(part 1 of 4)
# Autodesk Inventor assembly: ASSEMBLY_Main
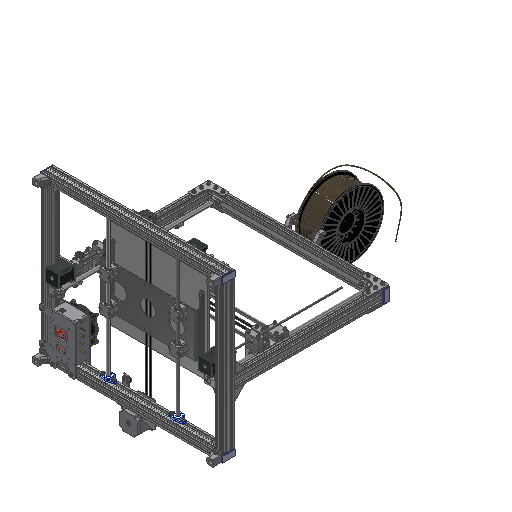
[picture p0: Inventor's stored thumbnail of the model, 512x512]
Saved by Autodesk Inventor 2026.1 (Build 301233000, 233)
## iProperties
Created: 2017-05-10
Part Number: ASSEMBLY_Main
Material: Ogólny
Document SubType Name: Assembly
Designer: Andrzej
Author: Andrzej
## Documents named in this file (88)
- C:\Users\Andrzej\OneDrive\_DRIVE_SYNCH_FILES\__ BYTECHLAB PROJECTS\MECH - FDM 3D Printer - TREX-300\MCAD\1_REV1\ASSEMBLY_MAIN_REVA\ASSEMBLY_Main.iam
- C:\Users\Andrzej\OneDrive\_DRIVE_SYNCH_FILES\__ BYTECHLAB PROJECTS\MECH - FDM 3D Printer - TREX-300\MCAD\1_REV1\ASSEMBLY_MAIN_REVA\LC_ALU_3mm_Top_Beam_Mounting_Bracket.ipt
- C:\Users\Andrzej\OneDrive\_DRIVE_SYNCH_FILES\__ BYTECHLAB PROJECTS\MECH - FDM 3D Printer - TREX-300\MCAD\1_REV1\__COTS_PARTS\COTS_GENERIC_20x40mm_alu_extrusion_460mm.ipt
- C:\Users\Andrzej\OneDrive\_DRIVE_SYNCH_FILES\__ BYTECHLAB PROJECTS\MECH - FDM 3D Printer - TREX-300\MCAD\1_REV1\__COTS_PARTS\COTS_GENERIC_20x40mm_alu_extrusion_560mm.ipt
- C:\Users\Andrzej\OneDrive\_DRIVE_SYNCH_FILES\__ BYTECHLAB PROJECTS\MECH - FDM 3D Printer - TREX-300\MCAD\1_REV1\__COTS_PARTS\COTS_GENERIC_20x40_Alu_Extrusion_Endcap.ipt
- C:\Users\Andrzej\OneDrive\_DRIVE_SYNCH_FILES\__ BYTECHLAB PROJECTS\MECH - FDM 3D Printer - TREX-300\MCAD\1_REV1\__COTS_PARTS\COTS_GENERIC_20x20mm_Angle_Bracket.ipt
- C:\Users\Andrzej\OneDrive\_DRIVE_SYNCH_FILES\__ BYTECHLAB PROJECTS\MECH - FDM 3D Printer - TREX-300\MCAD\1_REV1\ASSEMBLY_MAIN_REVA\CUT_STEEL_12mmx495mm_Linear_Shaft.ipt
- C:\Users\Andrzej\OneDrive\_DRIVE_SYNCH_FILES\__ BYTECHLAB PROJECTS\MECH - FDM 3D Printer - TREX-300\MCAD\1_REV1\ASSEMBLY_MAIN_REVA\CUT_STEEL_10mmx457mm_Linear_Shaft.ipt
- C:\Users\Andrzej\OneDrive\_DRIVE_SYNCH_FILES\__ BYTECHLAB PROJECTS\MECH - FDM 3D Printer - TREX-300\MCAD\1_REV1\ASSEMBLY_MAIN_REVA\LCBN_STEEL_3mm_Y_Axis_Heatbed_Baseplate.ipt
- C:\Users\Andrzej\OneDrive\_DRIVE_SYNCH_FILES\__ BYTECHLAB PROJECTS\MECH - FDM 3D Printer - TREX-300\MCAD\1_REV1\ASSEMBLY_MAIN_REVA\CNCM_ALU_6mm_Heatbed.ipt
- C:\Users\Andrzej\OneDrive\_DRIVE_SYNCH_FILES\__ BYTECHLAB PROJECTS\MECH - FDM 3D Printer - TREX-300\MCAD\1_REV1\ASSEMBLY_MAIN_REVA\CUT_STEEL_10mmx516mm_Linear_Shaft.ipt
- C:\Users\Andrzej\OneDrive\_DRIVE_SYNCH_FILES\__ BYTECHLAB PROJECTS\MECH - FDM 3D Printer - TREX-300\MCAD\1_REV1\ASSEMBLY_MAIN_REVA\LCBN_ALU_2mm_Y_Axis_Motor_Mount.ipt
- C:\Users\Andrzej\OneDrive\_DRIVE_SYNCH_FILES\__ BYTECHLAB PROJECTS\MECH - FDM 3D Printer - TREX-300\MCAD\1_REV1\ASSEMBLY_MAIN_REVA\3DP_ABS_Feet.ipt
- C:\Users\Andrzej\OneDrive\_DRIVE_SYNCH_FILES\__ BYTECHLAB PROJECTS\MECH - FDM 3D Printer - TREX-300\MCAD\1_REV1\ASSEMBLY_MAIN_REVA\3DP_ABS_Feet_MIR.ipt
- C:\Users\Andrzej\OneDrive\_DRIVE_SYNCH_FILES\__ BYTECHLAB PROJECTS\MECH - FDM 3D Printer - TREX-300\MCAD\1_REV1\ASSEMBLY_MAIN_REVA\3DP_ABS_Z_Axis_Endstop_Mount.ipt
- C:\Users\Andrzej\OneDrive\_DRIVE_SYNCH_FILES\__ BYTECHLAB PROJECTS\MECH - FDM 3D Printer - TREX-300\MCAD\1_REV1\__COTS_PARTS\COTS_GENERIC_Endstop.ipt
- C:\Users\Andrzej\OneDrive\_DRIVE_SYNCH_FILES\__ BYTECHLAB PROJECTS\MECH - FDM 3D Printer - TREX-300\MCAD\1_REV1\ASSEMBLY_MAIN_REVA\CNCM_ALU_3mm_Y_Axis_Idler_Stiffener_Side.ipt
- C:\Users\Andrzej\OneDrive\_DRIVE_SYNCH_FILES\__ BYTECHLAB PROJECTS\MECH - FDM 3D Printer - TREX-300\MCAD\1_REV1\ASSEMBLY_MAIN_REVA\LCBN_ALU_3mm_Y_Axis_Idler_Stiffener_Top.ipt
- C:\Users\Andrzej\OneDrive\_DRIVE_SYNCH_FILES\__ BYTECHLAB PROJECTS\MECH - FDM 3D Printer - TREX-300\MCAD\1_REV1\ASSEMBLY_MAIN_REVA\3DP_ABS_Y_Axis_Endstop_Mount.ipt
- C:\Users\Andrzej\OneDrive\_DRIVE_SYNCH_FILES\__ BYTECHLAB PROJECTS\MECH - FDM 3D Printer - TREX-300\MCAD\1_REV1\__COTS_PARTS\COTS_GENERIC_Bearing_12x5x5.ipt
- C:\Users\Andrzej\OneDrive\_DRIVE_SYNCH_FILES\__ BYTECHLAB PROJECTS\MECH - FDM 3D Printer - TREX-300\MCAD\1_REV1\__COTS_PARTS\COTS_GENERIC_Y_Axis_Timing_Belt.ipt
- C:\Users\Andrzej\OneDrive\_DRIVE_SYNCH_FILES\__ BYTECHLAB PROJECTS\MECH - FDM 3D Printer - TREX-300\MCAD\1_REV1\ASSEMBLY_MAIN_REVA\3DP_ABS_Y_Axis_Linear_Bearing_Mount_Top.ipt
- C:\Users\Andrzej\OneDrive\_DRIVE_SYNCH_FILES\__ BYTECHLAB PROJECTS\MECH - FDM 3D Printer - TREX-300\MCAD\1_REV1\ASSEMBLY_MAIN_REVA\3DP_ABS_Y_Axis_Linear_Bearing_Mount_Bottom.ipt
- C:\Users\Andrzej\OneDrive\_DRIVE_SYNCH_FILES\__ BYTECHLAB PROJECTS\MECH - FDM 3D Printer - TREX-300\MCAD\1_REV1\ASSEMBLY_MAIN_REVA\3DP_ABS_Y_Axis_Belt_Mount_Spacer.ipt
- C:\Users\Andrzej\OneDrive\_DRIVE_SYNCH_FILES\__ BYTECHLAB PROJECTS\MECH - FDM 3D Printer - TREX-300\MCAD\1_REV1\ASSEMBLY_MAIN_REVA\LC_ALU_4mm_X_End_Motor_Side.ipt
- C:\Users\Andrzej\OneDrive\_DRIVE_SYNCH_FILES\__ BYTECHLAB PROJECTS\MECH - FDM 3D Printer - TREX-300\MCAD\1_REV1\ASSEMBLY_MAIN_REVA\3DP_ABS_X_Axis_Linear_Shaft_Clamp_Base.ipt
- C:\Users\Andrzej\OneDrive\_DRIVE_SYNCH_FILES\__ BYTECHLAB PROJECTS\MECH - FDM 3D Printer - TREX-300\MCAD\1_REV1\ASSEMBLY_MAIN_REVA\LC_ALU_4mm_X_End_Bearing_Side.ipt
- C:\Users\Andrzej\OneDrive\_DRIVE_SYNCH_FILES\__ BYTECHLAB PROJECTS\MECH - FDM 3D Printer - TREX-300\MCAD\1_REV1\ASSEMBLY_MAIN_REVA\3DP_ABS_X_Axis_Linear_Shaft_Clamp_Top.ipt
- C:\Users\Andrzej\OneDrive\_DRIVE_SYNCH_FILES\__ BYTECHLAB PROJECTS\MECH - FDM 3D Printer - TREX-300\MCAD\1_REV1\ASSEMBLY_MAIN_REVA\3DP_ABS_X_Axis_Linear_Shaft_Clamp_Bottom.ipt
- C:\Users\Andrzej\OneDrive\_DRIVE_SYNCH_FILES\__ BYTECHLAB PROJECTS\MECH - FDM 3D Printer - TREX-300\MCAD\1_REV1\ASSEMBLY_MAIN_REVA\3DP_PLA_Controller_Case_Bottom.ipt
- C:\Users\Andrzej\OneDrive\_DRIVE_SYNCH_FILES\__ BYTECHLAB PROJECTS\MECH - FDM 3D Printer - TREX-300\MCAD\1_REV1\ASSEMBLY_MAIN_REVA\3DP_PLA_Controller_Case_Side_Wall_Longer.ipt
- C:\Users\Andrzej\OneDrive\_DRIVE_SYNCH_FILES\__ BYTECHLAB PROJECTS\MECH - FDM 3D Printer - TREX-300\MCAD\1_REV1\ASSEMBLY_MAIN_REVA\3DP_PLA_Controller_Case_Side_Wall_Shorter.ipt
- C:\Users\Andrzej\OneDrive\_DRIVE_SYNCH_FILES\__ BYTECHLAB PROJECTS\MECH - FDM 3D Printer - TREX-300\MCAD\1_REV1\ASSEMBLY_MAIN_REVA\3DP_PLA_Controller_Case_Top.ipt
- C:\Users\Andrzej\OneDrive\_DRIVE_SYNCH_FILES\__ BYTECHLAB PROJECTS\MECH - FDM 3D Printer - TREX-300\MCAD\1_REV1\ASSEMBLY_MAIN_REVA\3DP_PLA_Controller_Case_Fan_Grill.ipt
- C:\Users\Andrzej\OneDrive\_DRIVE_SYNCH_FILES\__ BYTECHLAB PROJECTS\MECH - FDM 3D Printer - TREX-300\MCAD\1_REV1\ASSEMBLY_MAIN_REVA\3DP_PLA_Filament_Spool_Rollers.ipt
- C:\Users\Andrzej\OneDrive\_DRIVE_SYNCH_FILES\__ BYTECHLAB PROJECTS\MECH - FDM 3D Printer - TREX-300\MCAD\1_REV1\__COTS_PARTS\COTS_GENERIC_Bearing_19x5x6.ipt
- C:\Users\Andrzej\OneDrive\_DRIVE_SYNCH_FILES\__ BYTECHLAB PROJECTS\MECH - FDM 3D Printer - TREX-300\MCAD\1_REV1\__COTS_PARTS\COTS_GENERIC_1_75mm_Filament_Spool.ipt
- C:\Users\Andrzej\OneDrive\_DRIVE_SYNCH_FILES\__ BYTECHLAB PROJECTS\MECH - FDM 3D Printer - TREX-300\MCAD\1_REV1\ASSEMBLY_MAIN_REVA\3DP_ABS_X_Axis_Endstop_Mount.ipt
- C:\Users\Andrzej\OneDrive\_DRIVE_SYNCH_FILES\__ BYTECHLAB PROJECTS\MECH - FDM 3D Printer - TREX-300\MCAD\1_REV1\ASSEMBLY_MAIN_REVA\3DP_ABS_X_Axis_Linear_Shaft_Clamp_Bottom_With_Endstop_Screw.ipt
- C:\Users\Andrzej\OneDrive\_DRIVE_SYNCH_FILES\__ BYTECHLAB PROJECTS\MECH - FDM 3D Printer - TREX-300\MCAD\1_REV1\ASSEMBLY_MAIN_REVA\3DP_ABS_Z_Axis_Screw_Nut_Mount.ipt
- C:\Users\Andrzej\OneDrive\_DRIVE_SYNCH_FILES\__ BYTECHLAB PROJECTS\MECH - FDM 3D Printer - TREX-300\MCAD\1_REV1\__COTS_PARTS\COTS_GENERIC_M6x350mm_Z_Axis_Screw.ipt
- C:\Users\Andrzej\OneDrive\_DRIVE_SYNCH_FILES\__ BYTECHLAB PROJECTS\MECH - FDM 3D Printer - TREX-300\MCAD\1_REV1\__COTS_PARTS\COTS_GENERIC_Z_Axis_M6_Screw_Nut.ipt
- C:\Users\Andrzej\OneDrive\_DRIVE_SYNCH_FILES\__ BYTECHLAB PROJECTS\MECH - FDM 3D Printer - TREX-300\MCAD\1_REV1\ASSEMBLY_MAIN_REVA\LC_ALU_4mm_Z_Axis_Motor_Mount.ipt
- C:\Users\Andrzej\OneDrive\_DRIVE_SYNCH_FILES\__ BYTECHLAB PROJECTS\MECH - FDM 3D Printer - TREX-300\MCAD\1_REV1\ASSEMBLY_MAIN_REVA\3DP_ABS_Z_Axis_Screw_Coupler.ipt
- C:\Users\Andrzej\OneDrive\_DRIVE_SYNCH_FILES\__ BYTECHLAB PROJECTS\MECH - FDM 3D Printer - TREX-300\MCAD\1_REV1\__COTS_PARTS\COTS_GENERIC_MXL_Pulley_X_Axis.ipt
- C:\Users\Andrzej\OneDrive\_DRIVE_SYNCH_FILES\__ BYTECHLAB PROJECTS\MECH - FDM 3D Printer - TREX-300\MCAD\1_REV1\__COTS_PARTS\COTS_GENERIC_Bearing_13x4x5.ipt
- C:\Users\Andrzej\OneDrive\_DRIVE_SYNCH_FILES\__ BYTECHLAB PROJECTS\MECH - FDM 3D Printer - TREX-300\MCAD\1_REV1\ASSEMBLY_MAIN_REVA\3DP_ABS_Cable_Pipe_Mount.ipt
- C:\Users\Andrzej\OneDrive\_DRIVE_SYNCH_FILES\__ BYTECHLAB PROJECTS\MECH - FDM 3D Printer - TREX-300\MCAD\1_REV1\ASSEMBLY_MAIN_REVA\3DP_ABS_X_End_Bearing_Mount.ipt
- C:\Users\Andrzej\OneDrive\_DRIVE_SYNCH_FILES\__ BYTECHLAB PROJECTS\MECH - FDM 3D Printer - TREX-300\MCAD\1_REV1\__COTS_PARTS\COTS_GENERIC_X_Axis_Timing_Belt.ipt
- C:\Users\Andrzej\OneDrive\_DRIVE_SYNCH_FILES\__ BYTECHLAB PROJECTS\MECH - FDM 3D Printer - TREX-300\MCAD\1_REV1\ASSEMBLY_MAIN_REVA\3DP_ABS_X_Axis_Motor_Spacer.ipt
- C:\Users\Andrzej\OneDrive\_DRIVE_SYNCH_FILES\__ BYTECHLAB PROJECTS\MECH - FDM 3D Printer - TREX-300\MCAD\1_REV1\ASSEMBLY_X_AXIS_CARRIAGE_AND_EXTRUDER\ASSEMBLY_X_Axis_Carriage_and_Extruder_Belt_Gearbox.iam
- C:\Users\Andrzej\OneDrive\_DRIVE_SYNCH_FILES\__ BYTECHLAB PROJECTS\MECH - FDM 3D Printer - TREX-300\MCAD\1_REV1\__COTS_PARTS\COTS_GENERIC_RAMPS_14_Ardunio_Mega\COTS_GENERIC_RAMPS_14_Ardunio_Mega.iam
- C:\Users\Andrzej\OneDrive\_DRIVE_SYNCH_FILES\__ BYTECHLAB PROJECTS\MECH - FDM 3D Printer - TREX-300\MCAD\1_REV1\__COTS_PARTS\COTS_GENERIC_80mm_fan\COTS_GENERIC_80mm_fan.iam
- C:\Users\Andrzej\OneDrive\_DRIVE_SYNCH_FILES\__ BYTECHLAB PROJECTS\MECH - FDM 3D Printer - TREX-300\MCAD\1_REV1\__CONTENT_CENTER_PARTS\en-US\DIN 125-1  A\DIN 125 - A 5,3.ipt
- C:\Users\Andrzej\OneDrive\_DRIVE_SYNCH_FILES\__ BYTECHLAB PROJECTS\MECH - FDM 3D Printer - TREX-300\MCAD\1_REV1\__CONTENT_CENTER_PARTS\en-US\DIN 912\DIN 912 - M5 x 0,8 x 30 x 22.ipt
- C:\Users\Andrzej\OneDrive\_DRIVE_SYNCH_FILES\__ BYTECHLAB PROJECTS\MECH - FDM 3D Printer - TREX-300\MCAD\1_REV1\__CONTENT_CENTER_PARTS\en-US\DIN 912\DIN 912 - M5 x 0,8 x 50 x 22.ipt
- C:\Users\Andrzej\OneDrive\_DRIVE_SYNCH_FILES\__ BYTECHLAB PROJECTS\MECH - FDM 3D Printer - TREX-300\MCAD\1_REV1\__CONTENT_CENTER_PARTS\en-US\DIN 125-1  A\DIN 125 - A 3,2.ipt
- C:\Users\Andrzej\OneDrive\_DRIVE_SYNCH_FILES\__ BYTECHLAB PROJECTS\MECH - FDM 3D Printer - TREX-300\MCAD\1_REV1\__CONTENT_CENTER_PARTS\en-US\ISO 7380-1\ISO 7380-1 - M3 x 12.ipt
- C:\Users\Andrzej\OneDrive\_DRIVE_SYNCH_FILES\__ BYTECHLAB PROJECTS\MECH - FDM 3D Printer - TREX-300\MCAD\1_REV1\__CONTENT_CENTER_PARTS\en-US\ISO 7380-1\ISO 7380-1 - M3 x 30.ipt
- C:\Users\Andrzej\OneDrive\_DRIVE_SYNCH_FILES\__ BYTECHLAB PROJECTS\MECH - FDM 3D Printer - TREX-300\MCAD\1_REV1\__CONTENT_CENTER_PARTS\en-US\DIN 934\DIN 934 - M3 x 0,5.ipt
- C:\Users\Andrzej\OneDrive\_DRIVE_SYNCH_FILES\__ BYTECHLAB PROJECTS\MECH - FDM 3D Printer - TREX-300\MCAD\1_REV1\__CONTENT_CENTER_PARTS\en-US\ISO 7380-1\ISO 7380-1 - M3 x 20.ipt
- C:\Users\Andrzej\OneDrive\_DRIVE_SYNCH_FILES\__ BYTECHLAB PROJECTS\MECH - FDM 3D Printer - TREX-300\MCAD\1_REV1\__CONTENT_CENTER_PARTS\en-US\DIN 912\DIN 912 - M3 x 0,5 x 20 x 18,75.ipt
- C:\Users\Andrzej\OneDrive\_DRIVE_SYNCH_FILES\__ BYTECHLAB PROJECTS\MECH - FDM 3D Printer - TREX-300\MCAD\1_REV1\__CONTENT_CENTER_PARTS\en-US\DIN 125-1  A\DIN 125 - A 4,3.ipt
- C:\Users\Andrzej\OneDrive\_DRIVE_SYNCH_FILES\__ BYTECHLAB PROJECTS\MECH - FDM 3D Printer - TREX-300\MCAD\1_REV1\__CONTENT_CENTER_PARTS\en-US\DIN 912\DIN 912 - M4 x 0,7 x 30 x 20.ipt
- C:\Users\Andrzej\OneDrive\_DRIVE_SYNCH_FILES\__ BYTECHLAB PROJECTS\MECH - FDM 3D Printer - TREX-300\MCAD\1_REV1\__CONTENT_CENTER_PARTS\en-US\DIN 934\DIN 934 - M4 x 0,7.ipt
- C:\Users\Andrzej\OneDrive\_DRIVE_SYNCH_FILES\__ BYTECHLAB PROJECTS\MECH - FDM 3D Printer - TREX-300\MCAD\1_REV1\__COTS_PARTS\COTS_GENERIC_20x20_M3_Nut.ipt
- C:\Users\Andrzej\OneDrive\_DRIVE_SYNCH_FILES\__ BYTECHLAB PROJECTS\MECH - FDM 3D Printer - TREX-300\MCAD\1_REV1\__CONTENT_CENTER_PARTS\en-US\DIN 912\DIN 912 - M3 x 0,5 x 16 x 14,75.ipt
- C:\Users\Andrzej\OneDrive\_DRIVE_SYNCH_FILES\__ BYTECHLAB PROJECTS\MECH - FDM 3D Printer - TREX-300\MCAD\1_REV1\__CONTENT_CENTER_PARTS\en-US\DIN 912\DIN 912 - M5 x 0,8 x 25 x 23.ipt
- C:\Users\Andrzej\OneDrive\_DRIVE_SYNCH_FILES\__ BYTECHLAB PROJECTS\MECH - FDM 3D Printer - TREX-300\MCAD\1_REV1\__CONTENT_CENTER_PARTS\en-US\DIN 934\DIN 934 - M5 x 0,8.ipt
- C:\Users\Andrzej\OneDrive\_DRIVE_SYNCH_FILES\__ BYTECHLAB PROJECTS\MECH - FDM 3D Printer - TREX-300\MCAD\1_REV1\__CONTENT_CENTER_PARTS\en-US\DIN 912\DIN 912 - M5 x 0,8 x 8 x 6.ipt
- C:\Users\Andrzej\OneDrive\_DRIVE_SYNCH_FILES\__ BYTECHLAB PROJECTS\MECH - FDM 3D Printer - TREX-300\MCAD\1_REV1\__CONTENT_CENTER_PARTS\en-US\DIN 912\DIN 912 - M5 x 0,8 x 12 x 10.ipt
- C:\Users\Andrzej\OneDrive\_DRIVE_SYNCH_FILES\__ BYTECHLAB PROJECTS\MECH - FDM 3D Printer - TREX-300\MCAD\1_REV1\__CONTENT_CENTER_PARTS\en-US\DIN 912\DIN 912 - M3 x 0,5 x 8 x 6,75.ipt
- C:\Users\Andrzej\OneDrive\_DRIVE_SYNCH_FILES\__ BYTECHLAB PROJECTS\MECH - FDM 3D Printer - TREX-300\MCAD\1_REV1\__CONTENT_CENTER_PARTS\en-US\DIN 7991(2)\DIN 7991 - M3x8.ipt
- C:\Users\Andrzej\OneDrive\_DRIVE_SYNCH_FILES\__ BYTECHLAB PROJECTS\MECH - FDM 3D Printer - TREX-300\MCAD\1_REV1\__CONTENT_CENTER_PARTS\en-US\DIN 912\DIN 912 - M4 x 0,7 x 40 x 20.ipt
- C:\Users\Andrzej\OneDrive\_DRIVE_SYNCH_FILES\__ BYTECHLAB PROJECTS\MECH - FDM 3D Printer - TREX-300\MCAD\1_REV1\__COTS_PARTS\COTS_GENERIC_NEMA17_25mm_shaft.ipt
- C:\Users\Andrzej\OneDrive\_DRIVE_SYNCH_FILES\__ BYTECHLAB PROJECTS\MECH - FDM 3D Printer - TREX-300\MCAD\1_REV1\__COTS_PARTS\COTS_GENERIC_SHF12_Linear_Rail_Mount\COTS_GENERIC_SHF12_Linear_Rail_Mount.iam
- C:\Users\Andrzej\OneDrive\_DRIVE_SYNCH_FILES\__ BYTECHLAB PROJECTS\MECH - FDM 3D Printer - TREX-300\MCAD\1_REV1\__COTS_PARTS\COTS_GENERIC_SK12_Linear_Rail_Mount\COTS_GENERIC_SK12_Linear_Rail_Mount.iam
- C:\Users\Andrzej\OneDrive\_DRIVE_SYNCH_FILES\__ BYTECHLAB PROJECTS\MECH - FDM 3D Printer - TREX-300\MCAD\1_REV1\__COTS_PARTS\COTS_GENERIC_NEMA23_Stepper_Motor\COTS_GENERIC_NEMA23_Stepper_Motor.iam
- C:\Users\Andrzej\OneDrive\_DRIVE_SYNCH_FILES\__ BYTECHLAB PROJECTS\MECH - FDM 3D Printer - TREX-300\MCAD\1_REV1\__COTS_PARTS\COTS_GENERIC_LM10UU_10mm_Linear_Bearing.ipt
- C:\Users\Andrzej\OneDrive\_DRIVE_SYNCH_FILES\__ BYTECHLAB PROJECTS\MECH - FDM 3D Printer - TREX-300\MCAD\1_REV1\__COTS_PARTS\COTS_GENERIC_SMA12GUU_Linear_Bearing_Block.ipt
- C:\Users\Andrzej\OneDrive\_DRIVE_SYNCH_FILES\__ BYTECHLAB PROJECTS\MECH - FDM 3D Printer - TREX-300\MCAD\1_REV1\__COTS_PARTS\COTS_GENERIC_SHF10_Linear_Rail_Mount.ipt
- C:\Users\Andrzej\OneDrive\_DRIVE_SYNCH_FILES\__ BYTECHLAB PROJECTS\MECH - FDM 3D Printer - TREX-300\MCAD\1_REV1\__COTS_PARTS\COTS_GENERIC_22x5_Washer.ipt
- C:\Users\Andrzej\OneDrive\_DRIVE_SYNCH_FILES\__ BYTECHLAB PROJECTS\MECH - FDM 3D Printer - TREX-300\MCAD\1_REV1\__CONTENT_CENTER_PARTS\en-US\DIN 912\DIN 912 - M4 x 0,7 x 8 x 6,25.ipt
- C:\Users\Andrzej\OneDrive\_DRIVE_SYNCH_FILES\__ BYTECHLAB PROJECTS\MECH - FDM 3D Printer - TREX-300\MCAD\1_REV1\__CONTENT_CENTER_PARTS\en-US\DIN 912\DIN 912 - M4 x 0,7 x 10 x 8,25.ipt
- C:\Users\Andrzej\OneDrive\_DRIVE_SYNCH_FILES\__ BYTECHLAB PROJECTS\MECH - FDM 3D Printer - TREX-300\MCAD\1_REV1\__CONTENT_CENTER_PARTS\en-US\DIN 912\DIN 912 - M5 x 0,8 x 10 x 8.ipt
- C:\Users\Andrzej\OneDrive\_DRIVE_SYNCH_FILES\__ BYTECHLAB PROJECTS\MECH - FDM 3D Printer - TREX-300\MCAD\1_REV1\__CONTENT_CENTER_PARTS\en-US\DIN 912\DIN 912 - M3 x 0,5 x 10 x 8,75.ipt
- C:\Users\Andrzej\OneDrive\_DRIVE_SYNCH_FILES\__ BYTECHLAB PROJECTS\MECH - FDM 3D Printer - TREX-300\MCAD\1_REV1\__CONTENT_CENTER_PARTS\en-US\DIN 912\DIN 912 - M3 x 0,5 x 30 x 18.ipt
- C:\Users\Andrzej\OneDrive\_DRIVE_SYNCH_FILES\__ BYTECHLAB PROJECTS\MECH - FDM 3D Printer - TREX-300\MCAD\1_REV1\__CONTENT_CENTER_PARTS\en-US\ISO 10642(1)\ISO 10642 - M4 x  20.ipt
## Components (507 placed, 87 different names)
1. COTS_GENERIC_20x40mm_alu_extrusion_460mm:1 — Zestawiający:7, Równoległy:13, Równoległy:14, Zestawiający:9, Równoległy:17, Równoległy:18, Zestawiający:10, Równoległy:19, Równoległy:25, Równoległy:48, Zestawiający:28, Zestawiający:32, Zestawiający:34, Równoległy:52, Równoległy:53, Zestawiający:40, Równoległy:55, Równoległy:69, Równoległy:76, Zestawiający:152, Równoległy:129, Równoległy:134, Zestawiający:211, Równoległy:150, Zestawiający:232
2. COTS_GENERIC_20x40mm_alu_extrusion_460mm:2 — Zestawiający:8, Równoległy:15, Równoległy:16, Zestawiający:11, Równoległy:20, Równoległy:47, Zestawiający:27, Zestawiający:31, Zestawiający:33, Równoległy:51, Równoległy:54, Zestawiający:39, Równoległy:56, Zestawiający:64, Równoległy:71, Równoległy:73, Zestawiający:207, Równoległy:149
3. COTS_GENERIC_20x40mm_alu_extrusion_460mm:3 — Zestawiający:10, Równoległy:19, Zestawiający:12, Równoległy:21, Równoległy:22, Równoległy:25, Zestawiający:13, Równoległy:26, Równoległy:28, Zestawiający:24, Zestawiający:30, Równoległy:49, Równoległy:57, Zestawiający:84, Równoległy:81, Równoległy:136, Zestawiający:230, Zestawiający:231, Zestawiający:233, Zestawiający:234
4. COTS_GENERIC_20x40mm_alu_extrusion_460mm:4 — Zestawiający:11, Równoległy:20, Równoległy:23, Równoległy:24, Zestawiający:16, Równoległy:31, Równoległy:42, Zestawiający:26, Zestawiający:29, Równoległy:50, Równoległy:58
5. COTS_GENERIC_20x40mm_alu_extrusion_560mm:1 — Zestawiający:7, Równoległy:13, Równoległy:14, Zestawiający:8, Równoległy:15, Równoległy:16, Zestawiający:19, Zestawiający:21, Równoległy:34, Równoległy:35, Równoległy:43, Równoległy:44, Zestawiający:35, Zestawiający:36, Zestawiający:53, Zestawiający:54, Równoległy:59, Równoległy:60, Zestawiający:61, Zestawiający:62, Zestawiający:76, Równoległy:72, Zestawiający:82, Równoległy:75, Zestawiający:94, Równoległy:89, Równoległy:92, Równoległy:93, Równoległy:128, Równoległy:135
6. COTS_GENERIC_20x40mm_alu_extrusion_560mm:2 — Zestawiający:12, Równoległy:21, Równoległy:22, Równoległy:23, Równoległy:24, Zestawiający:14, Zestawiający:15, Równoległy:27, Równoległy:29, Równoległy:30, Równoległy:33, Zestawiający:17, Zestawiający:20, Równoległy:38, Równoległy:39, Równoległy:40, Równoległy:41, Zestawiający:41, Zestawiający:42, Zestawiający:47, Zestawiający:48, Zestawiający:164, Zestawiający:165, Zestawiający:176, Zestawiający:177, Równoległy:155, Mate:306, Mate:307, Flush:161, Flush:162, Mate:363, Mate:364
7. COTS_GENERIC_20x40mm_alu_extrusion_560mm:3 — Zestawiający:9, Równoległy:17, Równoległy:18, Zestawiający:18, Zestawiający:22, Równoległy:36, Równoległy:37, Równoległy:45, Równoległy:46, Zestawiający:37, Zestawiający:38, Zestawiający:55, Zestawiający:56, Równoległy:61, Równoległy:62, Zestawiający:79, Równoległy:70, Zestawiający:80, Zestawiający:81, Równoległy:74, Zestawiający:86, Zestawiający:87, Równoległy:84, Równoległy:85
8. LC_ALU_3mm_Top_Beam_Mounting_Bracket:1 — Zestawiający:13, Równoległy:28, Równoległy:29
9. LC_ALU_3mm_Top_Beam_Mounting_Bracket:2 — Zestawiający:14, Równoległy:26, Równoległy:27
10. LC_ALU_3mm_Top_Beam_Mounting_Bracket:3 — Zestawiający:15, Równoległy:30, Równoległy:31, Mate:328, Mate:329, Mate:330, Mate:331, Mate:332, Mate:333, Mate:334, Mate:335, Mate:336, Mate:337
11. LC_ALU_3mm_Top_Beam_Mounting_Bracket:4 — Zestawiający:16, Równoległy:33, Równoległy:42
12. COTS_GENERIC_20x40_Alu_Extrusion_Endcap:1 — Zestawiający:18, Równoległy:45, Równoległy:46
13. COTS_GENERIC_20x40_Alu_Extrusion_Endcap:2 — Zestawiający:17, Równoległy:40, Równoległy:41
14. COTS_GENERIC_20x40_Alu_Extrusion_Endcap:3 — Zestawiający:19, Równoległy:43, Równoległy:44
15. COTS_GENERIC_20x40_Alu_Extrusion_Endcap:4 — Zestawiający:20, Równoległy:38, Równoległy:39
16. COTS_GENERIC_20x40_Alu_Extrusion_Endcap:5 — Zestawiający:21, Równoległy:34, Równoległy:35
17. COTS_GENERIC_20x40_Alu_Extrusion_Endcap:6 — Zestawiający:22, Równoległy:36, Równoległy:37
18. COTS_GENERIC_20x20mm_Angle_Bracket:1 — Zestawiający:33, Zestawiający:37, Równoległy:54, Mate:499, Mate:521, Mate:522, Mate:524
19. COTS_GENERIC_20x20mm_Angle_Bracket:2 — Zestawiający:24, Równoległy:48, Zestawiający:218, Mate:475, Mate:483
20. COTS_GENERIC_20x20mm_Angle_Bracket:3 — Zestawiający:28, Zestawiający:30, Równoległy:49, Mate:479, Mate:487
21. COTS_GENERIC_20x20mm_Angle_Bracket:4 — Zestawiający:34, Zestawiający:38, Równoległy:53, Mate:501, Mate:502, Mate:504, Mate:523
22. COTS_GENERIC_20x20mm_Angle_Bracket:5 — Zestawiający:26, Równoległy:47, Zestawiający:217, Mate:473, Mate:474, Mate:476, Mate:481, Mate:482, Mate:484
23. COTS_GENERIC_20x20mm_Angle_Bracket:6 — Zestawiający:31, Zestawiający:36, Równoległy:51, Mate:497, Mate:498, Mate:500, Mate:525, Mate:526, Mate:528
24. COTS_GENERIC_20x20mm_Angle_Bracket:7 — Zestawiający:32, Zestawiający:35, Równoległy:52, Mate:503, Mate:527
25. COTS_GENERIC_20x20mm_Angle_Bracket:8 — Zestawiający:27, Zestawiający:29, Równoległy:50, Mate:477, Mate:478, Mate:480, Mate:485, Mate:486, Mate:488
26. COTS_GENERIC_SK12_Linear_Rail_Mount:1 [sub-assembly] — Zestawiający:40, Równoległy:55, Równoległy:57, Zestawiający:45, Mate:493, Mate:494, Mate:495, Mate:496
27. COTS_GENERIC_SK12_Linear_Rail_Mount:2 [sub-assembly] — Zestawiający:39, Równoległy:56, Równoległy:58, Zestawiający:43, Mate:489, Mate:490, Mate:491, Mate:492
28. COTS_GENERIC_SHF12_Linear_Rail_Mount:1 [sub-assembly] — Zestawiający:41, Zestawiający:44, Mate:363, Mate:369, Mate:371
29. COTS_GENERIC_SHF12_Linear_Rail_Mount:2 [sub-assembly] — Zestawiający:42, Zestawiający:46, Mate:364, Mate:365, Mate:366, Mate:367, Mate:368, Mate:370, Mate:372
30. CUT_STEEL_12mmx495mm_Linear_Shaft:1 — Zestawiający:45, Zestawiający:46, Zestawiający:47, Zestawiający:49, Zestawiający:50
31. CUT_STEEL_12mmx495mm_Linear_Shaft:2 — Zestawiający:43, Zestawiający:44, Zestawiający:48, Zestawiający:51, Zestawiający:52
32. COTS_GENERIC_SMA12GUU_Linear_Bearing_Block:1 — Zestawiający:52, Równoległy:66, Równoległy:67, Równoległy:79, Równoległy:113, Równoległy:114
33. COTS_GENERIC_SMA12GUU_Linear_Bearing_Block:2 — Zestawiający:50, Równoległy:65, Równoległy:67, Równoległy:79, Zestawiający:134, Równoległy:104, Równoległy:106, Równoległy:158
34. COTS_GENERIC_SMA12GUU_Linear_Bearing_Block:3 — Zestawiający:51, Równoległy:66, Równoległy:80, Zestawiający:143
35. COTS_GENERIC_SMA12GUU_Linear_Bearing_Block:4 — Zestawiający:49, Równoległy:65, Równoległy:80, Równoległy:105
36. COTS_GENERIC_RAMPS_14_Ardunio_Mega:1 [sub-assembly] — Zestawiający:156, Zestawiający:191
37. ASSEMBLY_X_Axis_Carriage_and_Extruder_Belt_Gearbox:1 [sub-assembly] — Zestawiający:141, Zestawiający:142
38. COTS_GENERIC_SHF10_Linear_Rail_Mount:1 — Zestawiający:54, Zestawiający:58, Równoległy:60, Mate:541, Mate:543
39. COTS_GENERIC_SHF10_Linear_Rail_Mount:2 — Zestawiający:53, Zestawiający:57, Równoległy:59, Mate:537, Mate:538, Mate:539, Mate:540, Mate:542, Mate:544
40. COTS_GENERIC_SHF10_Linear_Rail_Mount:3 — Zestawiający:55, Zestawiający:59, Równoległy:61, Mate:533, Mate:535
41. COTS_GENERIC_SHF10_Linear_Rail_Mount:4 — Zestawiający:56, Zestawiający:60, Równoległy:62, Mate:529, Mate:530, Mate:531, Mate:532, Mate:534, Mate:536
42. CUT_STEEL_10mmx457mm_Linear_Shaft:1 — Zestawiający:57, Zestawiający:60, Zestawiający:61, Zestawiający:63, Zestawiający:67, Zestawiający:68, Zestawiający:71
43. CUT_STEEL_10mmx457mm_Linear_Shaft:2 — Zestawiający:58, Zestawiający:59, Zestawiający:62, Zestawiający:63, Zestawiający:64, Zestawiający:65, Zestawiający:66, Zestawiający:72, Zestawiający:125
44. COTS_GENERIC_LM10UU_10mm_Linear_Bearing:1 — Zestawiający:66, Zestawiający:128
45. COTS_GENERIC_LM10UU_10mm_Linear_Bearing:2 — Zestawiający:65, Zestawiający:126
46. COTS_GENERIC_LM10UU_10mm_Linear_Bearing:3 — Zestawiający:67, Zestawiający:124, Zestawiający:127
47. COTS_GENERIC_LM10UU_10mm_Linear_Bearing:4 — Zestawiający:68, Zestawiający:129
48. LCBN_STEEL_3mm_Y_Axis_Heatbed_Baseplate:1 — Zestawiający:71, Zestawiający:72, Zestawiający:73, Równoległy:63, Równoległy:64, Zestawiający:108, Zestawiający:109, Zestawiający:110, Zestawiający:111, Zestawiający:112, Zestawiający:113, Zestawiający:114, Zestawiający:115, Zestawiający:116, Zestawiający:117, Zestawiający:118, Zestawiający:119, Zestawiający:130, Zestawiający:131, Zestawiający:132, Zestawiający:133, Równoległy:102, Równoległy:103, Mate:609, Mate:610, Mate:612, Mate:614, Mate:616, Mate:618, Mate:620, Mate:622, Mate:624, Mate:625, Insert:171, Insert:172
49. CNCM_ALU_6mm_Heatbed:1 — Zestawiający:73, Równoległy:63, Równoległy:64, Mate:641, Mate:642
50. CUT_STEEL_10mmx516mm_Linear_Shaft:1 — Zestawiający:139, Równoległy:111, Zestawiający:142, Zestawiający:192
51. CUT_STEEL_10mmx516mm_Linear_Shaft:2 — Zestawiający:140, Równoległy:112, Zestawiający:141
52. COTS_GENERIC_NEMA17_25mm_shaft:1 — Zestawiający:135, Zestawiający:225, Zestawiający:228, Zestawiający:242, Zestawiający:243, Równoległy:159, Równoległy:160
53. COTS_GENERIC_NEMA17_25mm_shaft:2 — Zestawiający:201, Zestawiający:202, Zestawiający:208, Zestawiający:224, Mate:436
54. COTS_GENERIC_NEMA17_25mm_shaft:3 — Zestawiający:199, Zestawiający:200, Zestawiający:212, Zestawiający:213, Zestawiający:223, Mate:435
55. LCBN_ALU_2mm_Y_Axis_Motor_Mount:1 — Zestawiający:76, Zestawiający:77, Zestawiający:78, Równoległy:68, Równoległy:92, Równoległy:93, Mate:567, Mate:568, Mate:569, Mate:570, Mate:571, Mate:572, Mate:573, Mate:574, Mate:575, Mate:577, Mate:579, Mate:581, Mate:583, Mate:584, Mate:585, Mate:586, Mate:587, Mate:588, Mate:589, Mate:590
56. COTS_GENERIC_NEMA23_Stepper_Motor:1 [sub-assembly] — Zestawiający:77, Zestawiający:78, Równoległy:68, Zestawiający:101, Zestawiający:102, Mate:576, Mate:578, Mate:580, Mate:582
57. 3DP_ABS_Feet:1 — Zestawiający:79, Równoległy:69, Równoległy:70, Mate:597, Mate:603
58. 3DP_ABS_Feet:3 — Zestawiający:80, Równoległy:71, Równoległy:72, Mate:593, Mate:594, Mate:596, Mate:598, Mate:600, Mate:607
59. 3DP_ABS_Feet_MIR:1 — Zestawiający:81, Równoległy:73, Równoległy:74, Mate:595, Mate:601, Mate:602, Mate:604, Mate:606, Mate:608
60. 3DP_ABS_Feet_MIR:2 — Zestawiający:82, Równoległy:75, Równoległy:76, Mate:599, Mate:605
61. 3DP_ABS_Z_Axis_Endstop_Mount:1 — Zestawiający:84, Równoległy:81, Zestawiający:85, Równoległy:82, Równoległy:83, Mate:401, Mate:402
62. COTS_GENERIC_Endstop:1 — Zestawiający:95, Równoległy:90, Równoległy:91
63. COTS_GENERIC_Endstop:2 — Zestawiający:193, Równoległy:140, Równoległy:141, Mate:286, Mate:287, Mate:288, Mate:290, Mate:291, Mate:292
64. COTS_GENERIC_Endstop:3 — Zestawiający:85, Równoległy:82, Równoległy:83
65. CNCM_ALU_3mm_Y_Axis_Idler_Stiffener_Side:1 — Zestawiający:86, Równoległy:84, Zestawiający:88, Równoległy:86, Zestawiający:89, Mate:547, Mate:559, Mate:560, Mate:561, Mate:562, Mate:563, Mate:565
66. CNCM_ALU_3mm_Y_Axis_Idler_Stiffener_Side:2 — Zestawiający:87, Równoległy:85, Zestawiający:90, Mate:545, Mate:546, Mate:548, Mate:551, Mate:552, Mate:553, Mate:554, Mate:555, Mate:557
67. LCBN_ALU_3mm_Y_Axis_Idler_Stiffener_Top:1 — Zestawiający:88, Równoległy:86, Zestawiający:89, Zestawiający:90, Zestawiający:107, Mate:549, Mate:550, Mate:556, Mate:558, Mate:564, Mate:566
68. 3DP_ABS_Y_Axis_Endstop_Mount:1 — Zestawiający:94, Równoległy:89, Zestawiający:95, Równoległy:90, Równoległy:91, Mate:591, Mate:592
69. COTS_GENERIC_Bearing_12x5x5:1 — Zestawiający:98, Zestawiający:100, Zestawiający:103
70. COTS_GENERIC_Bearing_12x5x5:2 — Zestawiający:98, Zestawiający:104
71. COTS_GENERIC_Y_Axis_Timing_Belt:1 — Zestawiający:100, Zestawiający:101, Zestawiający:102
72. COTS_GENERIC_22x5_Washer:1 — Zestawiający:104
73. COTS_GENERIC_22x5_Washer:2 — Zestawiający:103, Zestawiający:107
74. 3DP_ABS_Y_Axis_Linear_Bearing_Mount_Top:1 — Zestawiający:108, Zestawiający:112, Zestawiający:113, Zestawiający:123, Równoległy:94, Równoległy:95, Zestawiający:128
75. 3DP_ABS_Y_Axis_Linear_Bearing_Mount_Top:2 — Zestawiający:111, Zestawiający:118, Zestawiający:119, Zestawiający:121, Równoległy:98, Równoległy:99, Zestawiający:124, Zestawiający:127
76. 3DP_ABS_Y_Axis_Linear_Bearing_Mount_Top:3 — Zestawiający:110, Zestawiający:116, Zestawiający:117, Zestawiający:120, Równoległy:100, Równoległy:101, Zestawiający:129
77. 3DP_ABS_Y_Axis_Linear_Bearing_Mount_Top:4 — Zestawiający:109, Zestawiający:114, Zestawiający:115, Zestawiający:122, Równoległy:96, Równoległy:97, Zestawiający:125, Zestawiający:126
78. 3DP_ABS_Y_Axis_Linear_Bearing_Mount_Bottom:1 — Zestawiający:120, Równoległy:100, Równoległy:101, Mate:621, Mate:623, Mate:637, Mate:639
79. 3DP_ABS_Y_Axis_Linear_Bearing_Mount_Bottom:2 — Zestawiający:122, Równoległy:96, Równoległy:97, Mate:613, Mate:615, Mate:629, Mate:631
80. 3DP_ABS_Y_Axis_Linear_Bearing_Mount_Bottom:3 — Zestawiający:121, Równoległy:98, Równoległy:99, Mate:617, Mate:619, Mate:633, Mate:635
81. 3DP_ABS_Y_Axis_Linear_Bearing_Mount_Bottom:4 — Zestawiający:123, Równoległy:94, Równoległy:95, Mate:611, Mate:626, Mate:627, Mate:628, Mate:630, Mate:632, Mate:634, Mate:636, Mate:638, Mate:640
82. 3DP_ABS_Y_Axis_Belt_Mount_Spacer:1 — Zestawiający:130, Zestawiający:132, Równoległy:102
83. 3DP_ABS_Y_Axis_Belt_Mount_Spacer:2 — Zestawiający:131, Zestawiający:133, Równoległy:103
84. LC_ALU_4mm_X_End_Motor_Side:1 — Zestawiający:134, Zestawiający:135, Równoległy:104, Równoległy:105, Równoległy:106, Zestawiający:137, Zestawiający:138, Równoległy:107, Równoległy:108, Równoległy:109, Równoległy:110, Równoległy:142, Zestawiający:228, Mate:276, Mate:277, Mate:278, Mate:279, Mate:280, Mate:281, Mate:282, Mate:283, Mate:285
85. 3DP_ABS_X_Axis_Linear_Shaft_Clamp_Base:1 — Zestawiający:137, Równoległy:107, Równoległy:108, Zestawiający:140, Równoległy:112, Zestawiający:146, Równoległy:119, Równoległy:120
86. 3DP_ABS_X_Axis_Linear_Shaft_Clamp_Base:2 — Zestawiający:138, Równoległy:109, Równoległy:110, Zestawiający:139, Równoległy:111, Zestawiający:194, Równoległy:143, Równoległy:144
87. LC_ALU_4mm_X_End_Bearing_Side:1 — Zestawiający:143, Równoległy:113, Równoległy:114, Zestawiający:144, Zestawiający:145, Równoległy:115, Równoległy:116, Równoległy:117, Równoległy:118, Zestawiający:226, Zestawiający:237, Równoległy:156, Równoległy:157, Zestawiający:238, Zestawiający:239, Mate:303, Mate:305
88. 3DP_ABS_X_Axis_Linear_Shaft_Clamp_Base:3 — Zestawiający:144, Równoległy:116, Równoległy:118, Zestawiający:147, Równoległy:121, Równoległy:122
89. 3DP_ABS_X_Axis_Linear_Shaft_Clamp_Base:4 — Zestawiający:145, Równoległy:115, Równoległy:117, Zestawiający:149, Równoległy:123, Równoległy:124
90. 3DP_ABS_X_Axis_Linear_Shaft_Clamp_Top:1 — Zestawiający:147, Równoległy:121, Równoległy:122, Mate:256, Mate:258, Mate:260, Mate:262
91. 3DP_ABS_X_Axis_Linear_Shaft_Clamp_Top:2 — Zestawiający:146, Równoległy:119, Równoległy:120, Mate:244, Mate:245, Mate:246, Mate:247, Mate:248, Mate:249, Mate:250, Mate:251, Mate:253, Mate:255, Mate:257, Mate:259, Mate:261, Mate:263, Mate:265, Mate:267
92. 3DP_ABS_X_Axis_Linear_Shaft_Clamp_Bottom:2 — Zestawiający:149, Równoległy:123, Równoległy:124, Zestawiający:198, Równoległy:147, Równoległy:148, Mate:264, Mate:266
93. 3DP_PLA_Controller_Case_Bottom:1 — Zestawiający:152, Równoległy:128, Równoległy:129, Zestawiający:154, Równoległy:130, Równoległy:131, Zestawiający:155, Równoległy:132, Równoległy:133, Zestawiający:156, Zestawiający:191, Mate:513, Mate:514, Mate:515, Mate:516, Mate:517, Mate:518, Mate:519, Mate:520
94. COTS_GENERIC_80mm_fan:1 [sub-assembly] — Zestawiający:158, Zestawiający:159, Zestawiający:160, Zestawiający:161, Zestawiający:162, Zestawiający:163
95. 3DP_PLA_Controller_Case_Side_Wall_Longer:1 — Zestawiający:154, Równoległy:130, Równoległy:131, Zestawiający:157
96. 3DP_PLA_Controller_Case_Side_Wall_Shorter:1 — Zestawiający:155, Równoległy:132, Równoległy:133
97. 3DP_PLA_Controller_Case_Top:1 — Zestawiający:157, Równoległy:134, Równoległy:135, Zestawiający:158, Zestawiający:159, Zestawiający:160, Mate:462, Mate:464, Mate:466, Mate:468, Mate:505, Mate:506, Mate:507, Mate:508, Mate:509, Mate:510, Mate:511, Mate:512
98. 3DP_PLA_Controller_Case_Fan_Grill:1 — Zestawiający:161, Zestawiający:162, Zestawiający:163, Mate:453, Mate:454, Mate:455, Mate:456, Mate:457, Mate:458, Mate:459, Mate:460, Mate:461, Mate:463, Mate:465, Mate:467
99. 3DP_PLA_Filament_Spool_Rollers:1 — Zestawiający:165, Równoległy:136, Zestawiający:166, Zestawiający:167, Zestawiający:170, Zestawiający:171, Zestawiający:176, Mate:311, Mate:325, Mate:327
100. 3DP_PLA_Filament_Spool_Rollers:2 — Zestawiający:164, Zestawiający:168, Zestawiający:169, Zestawiający:172, Zestawiający:173, Zestawiający:177, Mate:308, Mate:309, Mate:311, Mate:317, Mate:319
101. COTS_GENERIC_Bearing_19x5x6:1 — Zestawiający:166, Zestawiający:170, Zestawiający:175, Mate:320, Mate:321, Mate:323, Mate:324
102. COTS_GENERIC_Bearing_19x5x6:2 — Zestawiający:167, Zestawiający:171, Zestawiający:174, Mate:322, Mate:326
103. COTS_GENERIC_Bearing_19x5x6:3 — Zestawiający:169, Zestawiający:173, Mate:314, Mate:318
104. COTS_GENERIC_Bearing_19x5x6:4 — Zestawiający:168, Zestawiający:172, Mate:312, Mate:313, Mate:315, Mate:316
105. COTS_GENERIC_1_75mm_Filament_Spool:1 — Zestawiający:174, Zestawiający:175
106. 3DP_ABS_X_Axis_Endstop_Mount:1 — Zestawiający:192, Zestawiający:193, Równoległy:140, Równoległy:141, Równoległy:142, Mate:289, Mate:293
107. 3DP_ABS_X_Axis_Linear_Shaft_Clamp_Bottom_With_Endstop_Screw:1 — Zestawiający:194, Równoległy:143, Równoległy:144, Zestawiający:197, Równoległy:145, Równoległy:146, Mate:252, Mate:254, Mate:294, Mate:295, Mate:296, Mate:297
108. 3DP_ABS_Z_Axis_Screw_Nut_Mount:1 — Zestawiający:197, Równoległy:145, Równoległy:146, Zestawiający:203, Zestawiający:204, Zestawiający:220, Mate:268, Mate:269, Mate:270, Mate:271, Mate:273, Mate:275
109. 3DP_ABS_Z_Axis_Screw_Nut_Mount:2 — Zestawiający:198, Równoległy:147, Równoległy:148, Zestawiający:205, Zestawiający:206, Zestawiający:219, Mate:272, Mate:274
110. COTS_GENERIC_M6x350mm_Z_Axis_Screw:1 — Zestawiający:199, Zestawiający:200, Zestawiający:220
111. COTS_GENERIC_M6x350mm_Z_Axis_Screw:2 — Zestawiający:201, Zestawiający:202, Zestawiający:219
112. COTS_GENERIC_Z_Axis_M6_Screw_Nut:1 — Zestawiający:203, Zestawiający:204
113. COTS_GENERIC_Z_Axis_M6_Screw_Nut:2 — Zestawiający:205, Zestawiający:206
114. LC_ALU_4mm_Z_Axis_Motor_Mount:1 — Zestawiający:211, Równoległy:150, Zestawiający:212, Zestawiający:213, Zestawiający:218, Angle:10, Mate:445, Mate:447, Mate:449, Mate:451, Mate:471
115. LC_ALU_4mm_Z_Axis_Motor_Mount:2 — Zestawiający:207, Równoległy:149, Zestawiający:208, Zestawiający:217, Angle:11, Mate:437, Mate:438, Mate:439, Mate:440, Mate:441, Mate:442, Mate:443, Mate:444, Mate:446, Mate:448, Mate:450, Mate:452, Mate:469, Mate:470, Mate:472
116. 3DP_ABS_Z_Axis_Screw_Coupler:1 — Zestawiający:221, Równoległy:153, Równoległy:154, Angle:11, Mate:411, Mate:413, Mate:415, Mate:417, Mate:427, Mate:429, Mate:431, Mate:433, Mate:436
117. 3DP_ABS_Z_Axis_Screw_Coupler:2 — Zestawiający:222, Równoległy:151, Równoległy:152, Angle:10, Mate:403, Mate:404, Mate:405, Mate:406, Mate:407, Mate:408, Mate:409, Mate:410, Mate:412, Mate:414, Mate:416, Mate:418, Mate:419, Mate:421, Mate:423, Mate:425, Mate:435
118. 3DP_ABS_Z_Axis_Screw_Coupler:3 — Zestawiający:222, Równoległy:151, Równoległy:152, Zestawiający:223, Mate:420, Mate:422, Mate:424, Mate:426, Mate:428, Mate:430, Mate:432, Mate:434
119. 3DP_ABS_Z_Axis_Screw_Coupler:4 — Zestawiający:221, Równoległy:153, Równoległy:154, Zestawiający:224
120. COTS_GENERIC_MXL_Pulley_X_Axis:1 — Zestawiający:225, Zestawiający:240, Zestawiający:241, Zestawiający:242
121. COTS_GENERIC_Bearing_13x4x5:1 — Zestawiający:226, Zestawiający:227, Zestawiający:236, Zestawiający:238, Zestawiający:239
122. COTS_GENERIC_Bearing_13x4x5:2 — Zestawiający:227, Zestawiający:236, Mate:300, Mate:304
123. 3DP_ABS_Cable_Pipe_Mount:1 — Zestawiający:231, Równoległy:155, Zestawiający:234, Mate:387, Mate:391, Mate:392, Mate:394
124. 3DP_ABS_Cable_Pipe_Mount:2 — Zestawiający:230, Zestawiający:232, Zestawiający:233, Mate:385, Mate:386, Mate:388, Mate:393
125. 3DP_ABS_X_End_Bearing_Mount:1 — Zestawiający:237, Równoległy:156, Równoległy:157, Mate:298, Mate:299, Mate:301, Mate:302
126. COTS_GENERIC_X_Axis_Timing_Belt:1 — Zestawiający:240, Zestawiający:241, Równoległy:158
127. 3DP_ABS_X_Axis_Motor_Spacer:1 — Zestawiający:243, Równoległy:159, Równoległy:160, Mate:284
128. DIN 934 - replaced by DIN EN 24032/28673/28674 M3:27 — Mate:639, Mate:640
129. DIN 934 - replaced by DIN EN 24032/28673/28674 M3:26 — Mate:637, Mate:638
130. DIN 934 - replaced by DIN EN 24032/28673/28674 M3:25 — Mate:635, Mate:636
131. DIN 934 - replaced by DIN EN 24032/28673/28674 M3:24 — Mate:633, Mate:634
132. DIN 934 - replaced by DIN EN 24032/28673/28674 M3:23 — Mate:631, Mate:632
133. DIN 934 - replaced by DIN EN 24032/28673/28674 M3:22 — Mate:629, Mate:630
134. DIN 934 - replaced by DIN EN 24032/28673/28674 M3:21 — Mate:627, Mate:628
135. DIN 912 - replaced by DIN EN ISO 4762 M3 x 30:8 — Mate:623, Mate:624
136. DIN 912 - replaced by DIN EN ISO 4762 M3 x 30:7 — Mate:621, Mate:622
137. DIN 912 - replaced by DIN EN ISO 4762 M3 x 30:6 — Mate:619, Mate:620
138. DIN 912 - replaced by DIN EN ISO 4762 M3 x 30:5 — Mate:617, Mate:618
139. DIN 912 - replaced by DIN EN ISO 4762 M3 x 30:4 — Mate:615, Mate:616
140. DIN 912 - replaced by DIN EN ISO 4762 M3 x 30:3 — Mate:613, Mate:614
141. DIN 912 - replaced by DIN EN ISO 4762 M3 x 30:2 — Mate:611, Mate:612
142. DIN 934 - replaced by DIN EN 24032/28673/28674 M3:20 — Mate:625, Mate:626
143. DIN 912 - replaced by DIN EN ISO 4762 M3 x 30:1 — Mate:609, Mate:610
144. DIN 912 - replaced by DIN EN ISO 4762 M5 x 10:32 — Insert:170
145. DIN 912 - replaced by DIN EN ISO 4762 M5 x 10:31 — Insert:169
146. DIN 912 - replaced by DIN EN ISO 4762 M5 x 10:30 — Insert:168
147. DIN 125-1 A A 5,3:94 — Mate:607, Mate:608, Insert:170
148. DIN 125-1 A A 5,3:93 — Mate:605, Mate:606, Insert:169
149. DIN 125-1 A A 3,2:59 — Mate:581, Mate:582, Insert:157
150. DIN 125-1 A A 3,2:58 — Mate:579, Mate:580, Insert:156
151. DIN 125-1 A A 3,2:57 — Mate:577, Mate:578, Insert:155
152. DIN 912 - replaced by DIN EN ISO 4762 M3 x 16:8 — Insert:153
153. DIN 912 - replaced by DIN EN ISO 4762 M3 x 16:7 — Insert:152
154. DIN 912 - replaced by DIN EN ISO 4762 M3 x 16:6 — Insert:151
155. DIN 125-1 A A 3,2:56 — Mate:573, Mate:574, Insert:153
156. DIN 125-1 A A 3,2:55 — Mate:571, Mate:572, Insert:152